# Autodesk Inventor assembly: x_iddler
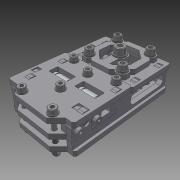
[picture p0: Inventor's stored thumbnail of the model, 180x180]
Saved by Autodesk Inventor 2014 (Build 180170000, 170)
## iProperties
Created: 2013-12-02
Part Number: x_iddler
Document SubType Name: Assembly
Designer: buben
Author: buben
## Documents named in this file (29)
- C:\Users\buben\Documents\GitHub\bacon\inventor files\assemblies\x_iddler.iam
- C:\Users\buben\Documents\GitHub\bacon\inventor files\printer parts\x_iddler_bottom.ipt
- C:\Users\buben\Documents\GitHub\bacon\inventor files\printer parts\x_iddler_wall_upper.ipt
- C:\Users\buben\Documents\GitHub\bacon\inventor files\printer parts\x_iddler_c_mount.ipt
- C:\Users\buben\Documents\GitHub\bacon\inventor files\printer parts\x_iddler_belt_bearing_mount.ipt
- C:\Users\buben\Documents\GitHub\bacon\inventor files\utils\washer_m6.ipt
- C:\Users\buben\Documents\Inventor\Content Center Files\R2014\en-US\ISO 4762(2)\ISO 4762 - M6 x 60ISO.ipt
- C:\Users\buben\Documents\Inventor\Content Center Files\R2014\en-US\ISO 7040\ISO 7040 - M6.ipt
- C:\Users\buben\Documents\GitHub\bacon\inventor files\utils\washer_m8.ipt
- C:\Users\buben\Documents\Inventor\Content Center Files\R2014\en-US\ISO 4762(2)\ISO 4762 - M8 x 60ISO.ipt
- C:\Users\buben\Documents\Inventor\Content Center Files\R2014\en-US\ISO 7040\ISO 7040 - M8.ipt
- C:\Users\buben\Documents\GitHub\bacon\inventor files\printer parts\x_motor_middle.ipt
- C:\Users\buben\Documents\GitHub\bacon\inventor files\printer parts\x_motor_smooth_rod_spacer.ipt
- C:\Users\buben\Documents\GitHub\bacon\inventor files\printer parts\x_iddler_wall_lower.ipt
- C:\Users\buben\Documents\GitHub\bacon\inventor files\printer parts\x_motor_lower_nut_stop.ipt
- C:\Users\buben\Documents\GitHub\bacon\inventor files\3rd party components\linear_bearing_8\Imported Components\LU8MM\LU8MM.iam
- C:\Users\buben\Documents\GitHub\bacon\inventor files\printer parts\x_motor_top.ipt
- C:\Users\buben\Documents\GitHub\bacon\inventor files\utils\washer_m5.ipt
- C:\Users\buben\Documents\Inventor\Content Center Files\R2014\en-US\ISO 4762(2)\ISO 4762 - M5 x 45ISO.ipt
- C:\Users\buben\Documents\Inventor\Content Center Files\R2014\en-US\ISO 7040\ISO 7040 - M5.ipt
- C:\Users\buben\Documents\GitHub\bacon\inventor files\printer parts\x_iddler_upper_nut_stop.ipt
- C:\Users\buben\Documents\GitHub\bacon\inventor files\utils\washer_m4.ipt
- C:\Users\buben\Documents\Inventor\Content Center Files\R2014\en-US\ISO 4762(2)\ISO 4762 - M4 x 20ISO.ipt
- C:\Users\buben\Documents\Inventor\Content Center Files\R2014\en-US\ISO 7040\ISO 7040 - M4.ipt
- C:\Users\buben\Documents\Inventor\Content Center Files\R2014\en-US\ISO 4032(2)\ISO 4032 - M5ISO.ipt
- C:\Users\buben\Documents\GitHub\bacon\inventor files\3rd party components\bearing_608\Imported Components\608RS\608RS.ipt
- C:\Users\buben\Documents\GitHub\bacon\inventor files\utils\belt_guide.ipt
- C:\Users\buben\Documents\GitHub\bacon\inventor files\utils\bearing_spacer_1.ipt
- C:\Users\buben\Documents\GitHub\bacon\inventor files\utils\bearing_spacer_2.ipt
## Components (75 placed, 28 different names)
1. x_iddler_bottom:1 — Flush:1, Mate:1, Flush:2, Mate:2, Mate:3, Mate:4, Mate:11, Mate:12, Mate:13, Mate:47, Mate:48, Mate:49, Mate:50, Mate:51, Mate:52, Mate:53, Mate:54, Mate:55, Mate:83, Mate:84, Mate:85, Mate:86, Mate:87, Mate:88, Mate:108
2. x_iddler_wall_upper:1 — Mate:2, Mate:3, Mate:4, Mate:5, Mate:6, Mate:7, Mate:56, Mate:57, Mate:58, Mate:107, Flush:4, Mate:136, Mate:137
3. x_iddler_c_mount:1 — Mate:5, Mate:6, Mate:7, Mate:8, Mate:9, Mate:10
4. x_iddler_belt_bearing_mount:1 — Mate:11, Mate:12, Mate:13, Mate:22, Mate:24, Mate:26, Mate:28, Mate:40, Mate:148
5. x_iddler_belt_bearing_mount:2 — Mate:8, Mate:9, Mate:10, Mate:14, Mate:15, Mate:16, Mate:17, Mate:18, Mate:19, Mate:20, Mate:21, Mate:38, Mate:39
6. CSN 02 1702 B B 6,4:1 — Mate:17, Mate:19, Insert:4
7. CSN 02 1702 B B 6,4:2 — Mate:14, Mate:21, Insert:2
8. CSN 02 1702 B B 6,4:3 — Mate:15, Mate:20, Insert:1
9. CSN 02 1702 B B 6,4:4 — Mate:16, Mate:18, Insert:3
10. ISO 4762 M6 x 60:1 — Insert:4, Mate:27, Mate:35
11. ISO 4762 M6 x 60:2 — Insert:2, Mate:25, Mate:33
12. ISO 4762 M6 x 60:3 — Insert:3, Mate:29, Mate:37
13. ISO 4762 M6 x 60:4 — Insert:1, Mate:23, Mate:31
14. CSN 02 1702 B B 6,4:5 — Mate:28, Mate:29, Mate:36
15. CSN 02 1702 B B 6,4:6 — Mate:26, Mate:27, Mate:34
16. CSN 02 1702 B B 6,4:7 — Mate:24, Mate:25, Mate:32
17. CSN 02 1702 B B 6,4:8 — Mate:22, Mate:23, Mate:30
18. DIN EN ISO 7040 M6:1 — Mate:32, Mate:33
19. DIN EN ISO 7040 M6:2 — Mate:30, Mate:31
20. DIN EN ISO 7040 M6:3 — Mate:34, Mate:35
21. DIN EN ISO 7040 M6:4 — Mate:36, Mate:37
22. CSN 02 1702 B B 8,4:1 — Mate:38, Mate:39, Insert:5
23. CSN 02 1702 B B 8,4:2 — Mate:40, Mate:41, Mate:42
24. ISO 4762 M8 x 60:1 — Insert:5, Mate:41, Mate:43, Mate:149, Mate:153
25. DIN EN ISO 7040 M8:1 — Mate:42, Mate:43
26. x_motor_smooth_rod_spacer:1 — Mate:50, Mate:51, Mate:52
27. x_motor_smooth_rod_spacer:2 — Mate:47, Mate:48, Mate:49
28. x_iddler_wall_lower:1 — Mate:53, Mate:54, Mate:55, Mate:60, Flush:3, Mate:67, Mate:70, Mate:109, Mate:110, Mate:111, Mate:112, Mate:133, Mate:134
29. x_motor_middle:1 — Mate:56, Mate:57, Mate:58, Mate:59, Mate:61, Mate:62, Mate:63, Mate:64, Mate:65, Mate:66
30. x_motor_lower_nut_stop:1 — Mate:59, Mate:60, Flush:3, Mate:117, Mate:118, Mate:135
31. LU8MM:1 [sub-assembly] — Mate:61, Mate:62, Mate:65
32. LU8MM:2 [sub-assembly] — Mate:63, Mate:64, Mate:66, Mate:68, Mate:69
33. x_motor_top:1 — Mate:67, Mate:68, Mate:69, Mate:70, Mate:71, Mate:72, Mate:73, Mate:74, Mate:75, Mate:76, Mate:77, Mate:78, Mate:79, Mate:80, Mate:81, Mate:82
34. CSN 02 1702 B B 5,3:1 — Mate:73, Mate:78, Insert:9
35. CSN 02 1702 B B 5,3:2 — Mate:72, Mate:80, Insert:6
36. CSN 02 1702 B B 5,3:3 — Mate:71, Mate:79, Insert:10
37. CSN 02 1702 B B 5,3:4 — Mate:76, Mate:77, Insert:11
38. CSN 02 1702 B B 5,3:5 — Mate:74, Mate:81, Insert:8
39. CSN 02 1702 B B 5,3:6 — Mate:75, Mate:82, Insert:7
40. ISO 4762 M5 x 45:1 — Insert:11, Mate:94, Mate:96
41. ISO 4762 M5 x 45:2 — Insert:10, Mate:92, Mate:106
42. ISO 4762 M5 x 45:3 — Insert:9, Mate:93, Mate:104
43. ISO 4762 M5 x 45:4 — Insert:8, Mate:90, Mate:102
44. ISO 4762 M5 x 45:5 — Insert:7, Mate:89, Mate:98
45. ISO 4762 M5 x 45:6 — Insert:6, Mate:91, Mate:100
46. CSN 02 1702 B B 5,3:7 — Mate:85, Mate:93, Mate:103
47. CSN 02 1702 B B 5,3:8 — Mate:86, Mate:89, Mate:97
48. CSN 02 1702 B B 5,3:9 — Mate:87, Mate:90, Mate:101
49. CSN 02 1702 B B 5,3:10 — Mate:88, Mate:91, Mate:99
50. CSN 02 1702 B B 5,3:11 — Mate:83, Mate:92, Mate:105
51. CSN 02 1702 B B 5,3:12 — Mate:84, Mate:94, Mate:95
52. DIN EN ISO 7040 M5:1 — Mate:95, Mate:96
53. DIN EN ISO 7040 M5:2 — Mate:97, Mate:98
54. DIN EN ISO 7040 M5:3 — Mate:99, Mate:100
55. DIN EN ISO 7040 M5:4 — Mate:103, Mate:104
56. DIN EN ISO 7040 M5:5 — Mate:105, Mate:106
57. DIN EN ISO 7040 M5:6 — Mate:101, Mate:102
58. x_iddler_upper_nut_stop:1 — Mate:107, Mate:108, Flush:4, Mate:138
59. CSN 02 1702 B B 4,3:3 — Mate:110, Mate:112, Insert:12
60. CSN 02 1702 B B 4,3:4 — Mate:109, Mate:111, Insert:13
61. ISO 4762 M4 x 20:3 — Insert:13, Mate:120, Mate:128
62. ISO 4762 M4 x 20:4 — Insert:12, Mate:119, Mate:126
63. CSN 02 1702 B B 4,3:5 — Mate:118, Mate:120, Mate:127
64. CSN 02 1702 B B 4,3:6 — Mate:117, Mate:119, Mate:125
65. DIN EN ISO 7040 M4:1 — Mate:127, Mate:128
66. DIN EN ISO 7040 M4:2 — Mate:125, Mate:126
67. ISO 4032 M5:1 — Mate:133, Mate:134, Mate:135
68. ISO 4032 M5:2 — Mate:136, Mate:137, Mate:138
69. 608RS:1 — Mate:139, Mate:140, Mate:143, Mate:144, Mate:145, Mate:152
70. belt_guide:1 — Mate:139, Mate:140, Mate:141, Mate:142
71. belt_guide:2 — Mate:141, Mate:142, Mate:143
72. CSN 02 1702 B B 8,4:3 — Mate:146, Mate:147, Mate:148
73. CSN 02 1702 B B 8,4:4 — Mate:150, Mate:151
74. bearing_spacer_1:1 — Mate:144, Mate:145, Mate:146, Mate:147, Mate:149
75. bearing_spacer_2:1 — Mate:150, Mate:151, Mate:152, Mate:153
## Relationships (155: Mate 138, Insert 13, Flush 4)
- Flush:1: x_iddler_bottom:1
- Mate:1: x_iddler_bottom:1
- Flush:2: x_iddler_bottom:1
- Mate:2: x_iddler_bottom:1 ↔ x_iddler_wall_upper:1
- Mate:3: x_iddler_bottom:1 ↔ x_iddler_wall_upper:1
- Mate:4: x_iddler_bottom:1 ↔ x_iddler_wall_upper:1
- Mate:5: x_iddler_wall_upper:1 ↔ x_iddler_c_mount:1
- Mate:6: x_iddler_wall_upper:1 ↔ x_iddler_c_mount:1
- Mate:7: x_iddler_wall_upper:1 ↔ x_iddler_c_mount:1
- Mate:8: x_iddler_c_mount:1 ↔ x_iddler_belt_bearing_mount:2
- Mate:9: x_iddler_c_mount:1 ↔ x_iddler_belt_bearing_mount:2
- Mate:10: x_iddler_c_mount:1 ↔ x_iddler_belt_bearing_mount:2
- Mate:11: x_iddler_bottom:1 ↔ x_iddler_belt_bearing_mount:1
- Mate:12: x_iddler_bottom:1 ↔ x_iddler_belt_bearing_mount:1
- Mate:13: x_iddler_bottom:1 ↔ x_iddler_belt_bearing_mount:1
- Mate:14: x_iddler_belt_bearing_mount:2 ↔ CSN 02 1702 B B 6,4:2
- Mate:15: x_iddler_belt_bearing_mount:2 ↔ CSN 02 1702 B B 6,4:3
- Mate:16: x_iddler_belt_bearing_mount:2 ↔ CSN 02 1702 B B 6,4:4
- Mate:17: x_iddler_belt_bearing_mount:2 ↔ CSN 02 1702 B B 6,4:1
- Mate:18: x_iddler_belt_bearing_mount:2 ↔ CSN 02 1702 B B 6,4:4
- Mate:19: x_iddler_belt_bearing_mount:2 ↔ CSN 02 1702 B B 6,4:1
- Mate:20: x_iddler_belt_bearing_mount:2 ↔ CSN 02 1702 B B 6,4:3
- Mate:21: x_iddler_belt_bearing_mount:2 ↔ CSN 02 1702 B B 6,4:2
- Insert:1: CSN 02 1702 B B 6,4:3 ↔ ISO 4762 M6 x 60:4
- Insert:2: CSN 02 1702 B B 6,4:2 ↔ ISO 4762 M6 x 60:2
- Insert:3: CSN 02 1702 B B 6,4:4 ↔ ISO 4762 M6 x 60:3
- Insert:4: CSN 02 1702 B B 6,4:1 ↔ ISO 4762 M6 x 60:1
- Mate:22: x_iddler_belt_bearing_mount:1 ↔ CSN 02 1702 B B 6,4:8
- Mate:23: ISO 4762 M6 x 60:4 ↔ CSN 02 1702 B B 6,4:8
- Mate:24: x_iddler_belt_bearing_mount:1 ↔ CSN 02 1702 B B 6,4:7
- Mate:25: ISO 4762 M6 x 60:2 ↔ CSN 02 1702 B B 6,4:7
- Mate:26: x_iddler_belt_bearing_mount:1 ↔ CSN 02 1702 B B 6,4:6
- Mate:27: ISO 4762 M6 x 60:1 ↔ CSN 02 1702 B B 6,4:6
- Mate:28: x_iddler_belt_bearing_mount:1 ↔ CSN 02 1702 B B 6,4:5
- Mate:29: ISO 4762 M6 x 60:3 ↔ CSN 02 1702 B B 6,4:5
- Mate:30: CSN 02 1702 B B 6,4:8 ↔ DIN EN ISO 7040 M6:2
- Mate:31: ISO 4762 M6 x 60:4 ↔ DIN EN ISO 7040 M6:2
- Mate:32: CSN 02 1702 B B 6,4:7 ↔ DIN EN ISO 7040 M6:1
- Mate:33: ISO 4762 M6 x 60:2 ↔ DIN EN ISO 7040 M6:1
- Mate:34: CSN 02 1702 B B 6,4:6 ↔ DIN EN ISO 7040 M6:3
- Mate:35: ISO 4762 M6 x 60:1 ↔ DIN EN ISO 7040 M6:3
- Mate:36: CSN 02 1702 B B 6,4:5 ↔ DIN EN ISO 7040 M6:4
- Mate:37: ISO 4762 M6 x 60:3 ↔ DIN EN ISO 7040 M6:4
- Mate:38: x_iddler_belt_bearing_mount:2 ↔ CSN 02 1702 B B 8,4:1
- Mate:39: x_iddler_belt_bearing_mount:2 ↔ CSN 02 1702 B B 8,4:1
- Insert:5: CSN 02 1702 B B 8,4:1 ↔ ISO 4762 M8 x 60:1
- Mate:40: x_iddler_belt_bearing_mount:1 ↔ CSN 02 1702 B B 8,4:2
- Mate:41: CSN 02 1702 B B 8,4:2 ↔ ISO 4762 M8 x 60:1
- Mate:42: CSN 02 1702 B B 8,4:2 ↔ DIN EN ISO 7040 M8:1
- Mate:43: ISO 4762 M8 x 60:1 ↔ DIN EN ISO 7040 M8:1
- Mate:47: x_iddler_bottom:1 ↔ x_motor_smooth_rod_spacer:2
- Mate:48: x_iddler_bottom:1 ↔ x_motor_smooth_rod_spacer:2
- Mate:49: x_iddler_bottom:1 ↔ x_motor_smooth_rod_spacer:2
- Mate:50: x_iddler_bottom:1 ↔ x_motor_smooth_rod_spacer:1
- Mate:51: x_iddler_bottom:1 ↔ x_motor_smooth_rod_spacer:1
- Mate:52: x_iddler_bottom:1 ↔ x_motor_smooth_rod_spacer:1
- Mate:53: x_iddler_bottom:1 ↔ x_iddler_wall_lower:1
- Mate:54: x_iddler_bottom:1 ↔ x_iddler_wall_lower:1
- Mate:55: x_iddler_bottom:1 ↔ x_iddler_wall_lower:1
- Mate:56: x_iddler_wall_upper:1 ↔ x_motor_middle:1
- Mate:57: x_iddler_wall_upper:1 ↔ x_motor_middle:1
- Mate:58: x_iddler_wall_upper:1 ↔ x_motor_middle:1
- Mate:59: x_motor_middle:1 ↔ x_motor_lower_nut_stop:1
- Mate:60: x_iddler_wall_lower:1 ↔ x_motor_lower_nut_stop:1
- Flush:3: x_iddler_wall_lower:1 ↔ x_motor_lower_nut_stop:1
- Mate:61 (7.5 mm): x_motor_middle:1 ↔ LU8MM:1
- Mate:62 (7.5 mm): x_motor_middle:1 ↔ LU8MM:1
- Mate:63 (7.5 mm): x_motor_middle:1 ↔ LU8MM:2
- Mate:64 (7.5 mm): x_motor_middle:1 ↔ LU8MM:2
- Mate:65 (0.5 mm): x_motor_middle:1 ↔ LU8MM:1
- Mate:66 (0.5 mm): x_motor_middle:1 ↔ LU8MM:2
- Mate:67: x_iddler_wall_lower:1 ↔ x_motor_top:1
- Mate:68 (7.5 mm): LU8MM:2 ↔ x_motor_top:1
- Mate:69 (7.5 mm): LU8MM:2 ↔ x_motor_top:1
- Mate:70: x_iddler_wall_lower:1 ↔ x_motor_top:1
- Mate:71: x_motor_top:1 ↔ CSN 02 1702 B B 5,3:3
- Mate:72: x_motor_top:1 ↔ CSN 02 1702 B B 5,3:2
- Mate:73: x_motor_top:1 ↔ CSN 02 1702 B B 5,3:1
- Mate:74: x_motor_top:1 ↔ CSN 02 1702 B B 5,3:5
- Mate:75: x_motor_top:1 ↔ CSN 02 1702 B B 5,3:6
- Mate:76: x_motor_top:1 ↔ CSN 02 1702 B B 5,3:4
- Mate:77: x_motor_top:1 ↔ CSN 02 1702 B B 5,3:4
- Mate:78: x_motor_top:1 ↔ CSN 02 1702 B B 5,3:1
- Mate:79: x_motor_top:1 ↔ CSN 02 1702 B B 5,3:3
- Mate:80: x_motor_top:1 ↔ CSN 02 1702 B B 5,3:2
- Mate:81: x_motor_top:1 ↔ CSN 02 1702 B B 5,3:5
- Mate:82: x_motor_top:1 ↔ CSN 02 1702 B B 5,3:6
- Insert:6: CSN 02 1702 B B 5,3:2 ↔ ISO 4762 M5 x 45:6
- Insert:7: CSN 02 1702 B B 5,3:6 ↔ ISO 4762 M5 x 45:5
- Insert:8: CSN 02 1702 B B 5,3:5 ↔ ISO 4762 M5 x 45:4
- Insert:9: CSN 02 1702 B B 5,3:1 ↔ ISO 4762 M5 x 45:3
- Insert:10: CSN 02 1702 B B 5,3:3 ↔ ISO 4762 M5 x 45:2
- Insert:11: CSN 02 1702 B B 5,3:4 ↔ ISO 4762 M5 x 45:1
- Mate:83: x_iddler_bottom:1 ↔ CSN 02 1702 B B 5,3:11
- Mate:84: x_iddler_bottom:1 ↔ CSN 02 1702 B B 5,3:12
- Mate:85: x_iddler_bottom:1 ↔ CSN 02 1702 B B 5,3:7
- Mate:86: x_iddler_bottom:1 ↔ CSN 02 1702 B B 5,3:8
- Mate:87: x_iddler_bottom:1 ↔ CSN 02 1702 B B 5,3:9
- Mate:88: x_iddler_bottom:1 ↔ CSN 02 1702 B B 5,3:10
- Mate:89: ISO 4762 M5 x 45:5 ↔ CSN 02 1702 B B 5,3:8
- Mate:90: ISO 4762 M5 x 45:4 ↔ CSN 02 1702 B B 5,3:9
- Mate:91: ISO 4762 M5 x 45:6 ↔ CSN 02 1702 B B 5,3:10
- Mate:92: ISO 4762 M5 x 45:2 ↔ CSN 02 1702 B B 5,3:11
- Mate:93: ISO 4762 M5 x 45:3 ↔ CSN 02 1702 B B 5,3:7
- Mate:94: ISO 4762 M5 x 45:1 ↔ CSN 02 1702 B B 5,3:12
- Mate:95: CSN 02 1702 B B 5,3:12 ↔ DIN EN ISO 7040 M5:1
- Mate:96: ISO 4762 M5 x 45:1 ↔ DIN EN ISO 7040 M5:1
- Mate:97: CSN 02 1702 B B 5,3:8 ↔ DIN EN ISO 7040 M5:2
- Mate:98: ISO 4762 M5 x 45:5 ↔ DIN EN ISO 7040 M5:2
- Mate:99: CSN 02 1702 B B 5,3:10 ↔ DIN EN ISO 7040 M5:3
- Mate:100: ISO 4762 M5 x 45:6 ↔ DIN EN ISO 7040 M5:3
- Mate:101: CSN 02 1702 B B 5,3:9 ↔ DIN EN ISO 7040 M5:6
- Mate:102: ISO 4762 M5 x 45:4 ↔ DIN EN ISO 7040 M5:6
- Mate:103: CSN 02 1702 B B 5,3:7 ↔ DIN EN ISO 7040 M5:4
- Mate:104: ISO 4762 M5 x 45:3 ↔ DIN EN ISO 7040 M5:4
- Mate:105: CSN 02 1702 B B 5,3:11 ↔ DIN EN ISO 7040 M5:5
- Mate:106: ISO 4762 M5 x 45:2 ↔ DIN EN ISO 7040 M5:5
- Mate:107: x_iddler_wall_upper:1 ↔ x_iddler_upper_nut_stop:1
- Mate:108: x_iddler_bottom:1 ↔ x_iddler_upper_nut_stop:1
- Flush:4: x_iddler_wall_upper:1 ↔ x_iddler_upper_nut_stop:1
- Mate:109: x_iddler_wall_lower:1 ↔ CSN 02 1702 B B 4,3:4
- Mate:110: x_iddler_wall_lower:1 ↔ CSN 02 1702 B B 4,3:3
- Mate:111: x_iddler_wall_lower:1 ↔ CSN 02 1702 B B 4,3:4
- Mate:112: x_iddler_wall_lower:1 ↔ CSN 02 1702 B B 4,3:3
- Insert:12: CSN 02 1702 B B 4,3:3 ↔ ISO 4762 M4 x 20:4
- Insert:13: CSN 02 1702 B B 4,3:4 ↔ ISO 4762 M4 x 20:3
- Mate:117: x_motor_lower_nut_stop:1 ↔ CSN 02 1702 B B 4,3:6
- Mate:118: x_motor_lower_nut_stop:1 ↔ CSN 02 1702 B B 4,3:5
- Mate:119: ISO 4762 M4 x 20:4 ↔ CSN 02 1702 B B 4,3:6
- Mate:120: ISO 4762 M4 x 20:3 ↔ CSN 02 1702 B B 4,3:5
- Mate:125: CSN 02 1702 B B 4,3:6 ↔ DIN EN ISO 7040 M4:2
- Mate:126: ISO 4762 M4 x 20:4 ↔ DIN EN ISO 7040 M4:2
- Mate:127: CSN 02 1702 B B 4,3:5 ↔ DIN EN ISO 7040 M4:1
- Mate:128: ISO 4762 M4 x 20:3 ↔ DIN EN ISO 7040 M4:1
- Mate:133: x_iddler_wall_lower:1 ↔ ISO 4032 M5:1
- Mate:134: x_iddler_wall_lower:1 ↔ ISO 4032 M5:1
- Mate:135: x_motor_lower_nut_stop:1 ↔ ISO 4032 M5:1
- Mate:136: x_iddler_wall_upper:1 ↔ ISO 4032 M5:2
- Mate:137: x_iddler_wall_upper:1 ↔ ISO 4032 M5:2
- Mate:138: x_iddler_upper_nut_stop:1 ↔ ISO 4032 M5:2
- Mate:139: 608RS:1 ↔ belt_guide:1
- Mate:140: 608RS:1 ↔ belt_guide:1
- Mate:141: belt_guide:1 ↔ belt_guide:2
- Mate:142: belt_guide:1 ↔ belt_guide:2
- Mate:143: 608RS:1 ↔ belt_guide:2
- Mate:144: 608RS:1 ↔ bearing_spacer_1:1
- Mate:145: 608RS:1 ↔ bearing_spacer_1:1
- Mate:146: CSN 02 1702 B B 8,4:3 ↔ bearing_spacer_1:1
- Mate:147: CSN 02 1702 B B 8,4:3 ↔ bearing_spacer_1:1
- Mate:148: x_iddler_belt_bearing_mount:1 ↔ CSN 02 1702 B B 8,4:3
- Mate:149: ISO 4762 M8 x 60:1 ↔ bearing_spacer_1:1
- Mate:150: CSN 02 1702 B B 8,4:4 ↔ bearing_spacer_2:1
- Mate:151: CSN 02 1702 B B 8,4:4 ↔ bearing_spacer_2:1
- Mate:152: 608RS:1 ↔ bearing_spacer_2:1
- Mate:153: ISO 4762 M8 x 60:1 ↔ bearing_spacer_2:1
